# Autodesk Inventor assembly: my gtx 1070 waterblock
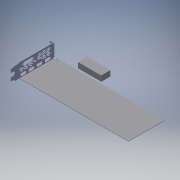
[picture p0: Inventor's stored thumbnail of the model, 180x180]
Saved by Autodesk Inventor 2018 (Build 220112000, 112)
## iProperties
Created: 2018-06-21
Part Number: my gtx 1070 waterblock
Document SubType Name: Assembly
Designer: John Viljoen
Author: John Viljoen
## Documents named in this file (4)
- C:\Users\John Viljoen\Documents\Inventor\computer project\my gtx 1070\my gtx 1070 waterblock.iam
- C:\Users\John Viljoen\Documents\Inventor\computer project\my gtx 1070\GTX 1070 Bracket.ipt
- C:\Users\John Viljoen\Documents\Inventor\computer project\my gtx 1070\gtx 1070 pcb.ipt
- C:\Users\John Viljoen\Documents\Inventor\computer project\my gtx 1070\waterblock connector.ipt
## Components (3 placed, 3 different names)
1. GTX 1070 Bracket:1 — Flush:1, Mate:1, Mate:2, Mate:3
2. gtx 1070 pcb:1 — Flush:1, Mate:1, Mate:2, Mate:4, Mate:5
3. waterblock connector:1 — Mate:3, Mate:4, Mate:5
## Relationships (6: Mate 5, Flush 1)
- Flush:1 (-5 mm): GTX 1070 Bracket:1 ↔ gtx 1070 pcb:1
- Mate:1 (2 mm): GTX 1070 Bracket:1 ↔ gtx 1070 pcb:1
- Mate:2: GTX 1070 Bracket:1 ↔ gtx 1070 pcb:1
- Mate:3 (60 mm): GTX 1070 Bracket:1 ↔ waterblock connector:1
- Mate:4: gtx 1070 pcb:1 ↔ waterblock connector:1
- Mate:5 (5 mm): gtx 1070 pcb:1 ↔ waterblock connector:1
